# Autodesk Inventor assembly: y-Max Endstop for 4040 - Assembly
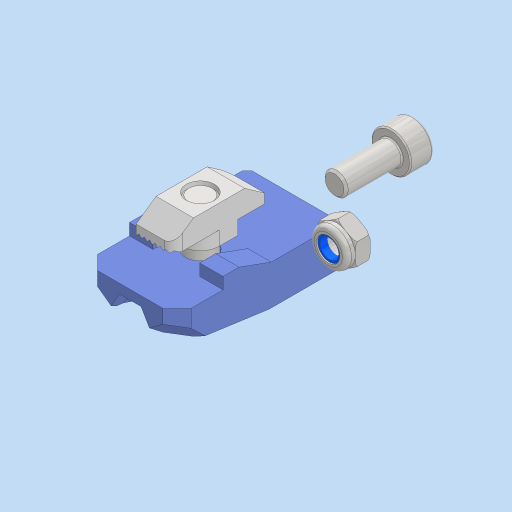
[picture p0: Inventor's stored thumbnail of the model, 512x512]
Saved by Autodesk Inventor 2023.2 (Build 272271000, 271)
## iProperties
Created: 2023-11-28
Part Number: y-Max Endstop for 4040 - Assembly
Document SubType Name: Assembly
Designer: Nils Bade
Author: Nils Bade
## Documents named in this file (7)
- C:\Users\nilsb\Documents\Inventor\Projektarbeit-Bade\RatRig_Bade\y-Max Endstop for 4040 - Assembly.iam
- C:\Users\nilsb\Documents\Inventor\Projektarbeit-Bade\RatRig_modified\y-Max Endstop Block for 4040.ipt
- C:\Users\nilsb\Documents\Inventor\Projektarbeit-Bade\RatRig_modified\T-NUT - DropIn 4040 SERIES - M6.ipt
- C:\Users\nilsb\Documents\Inventor\Projektarbeit-Bade\Schrauben\Cap Head Screw M6x12 v2.ipt
- C:\Users\nilsb\Documents\Inventor\Projektarbeit-Bade\Schrauben\Cap Head Screw M5x12 v2.ipt
- C:\Users\nilsb\Documents\Inventor\Projektarbeit-Bade\RatRig_Standards\Hex Locking Nut - M5 v2.ipt
- C:\Users\nilsb\Documents\Inventor\Projektarbeit-Bade\Schrauben\Cap Head Screw M3x12 v2.ipt
## Components (7 placed, 6 different names)
1. y-Max Endstop Block for 4040:1 — Passend:1, Passend:2, Winkel:1, Passend:3, Passend:4
2. T-NUT - DROP IN TYPE FOR 40 SERIES - M6:1 — Passend:1, Passend:2, Winkel:1
3. Cap Head Screw M6x12 v2:1 — Passend:3, Passend:4
4. Cap Head Screw M5x12 v2:1
5. Hex Locking Nut - M5 v2:1
6. Cap Head Screw M3x12 v2:1
7. Cap Head Screw M3x12 v2:2
## Relationships (5: Mate 4, Angle 1)
- Passend:1 [Mate]: y-Max Endstop Block for 4040:1 ↔ T-NUT - DROP IN TYPE FOR 40 SERIES - M6:1
- Passend:2 [Mate] (5.5 mm): y-Max Endstop Block for 4040:1 ↔ T-NUT - DROP IN TYPE FOR 40 SERIES - M6:1
- Winkel:1 [Angle] (0 deg): y-Max Endstop Block for 4040:1 ↔ T-NUT - DROP IN TYPE FOR 40 SERIES - M6:1
- Passend:3 [Mate]: y-Max Endstop Block for 4040:1 ↔ Cap Head Screw M6x12 v2:1
- Passend:4 [Mate]: y-Max Endstop Block for 4040:1 ↔ Cap Head Screw M6x12 v2:1
